# Autodesk Inventor assembly: Rwing
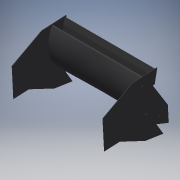
[picture p0: Inventor's stored thumbnail of the model, 180x180]
Saved by Autodesk Inventor 2018.2 (Build 222227000, 227)
## iProperties
Created: 2017-12-28
Part Number: Rwing
Material: 一般
Document SubType Name: Assembly
Designer: formula
Author: formula
## Documents named in this file (5)
- Z:\各班フォルダ\2018\ボディ\カウル\AeroCAD2018\CAD\Inventor\解析用CAD\R-wing\Rwing.iam
- Z:\各班フォルダ\2018\ボディ\カウル\AeroCAD2018\CAD\Inventor\解析用CAD\R-wing\parts\main_flap\parts\styro_50_main_center.ipt
- Z:\各班フォルダ\2018\ボディ\カウル\AeroCAD2018\CAD\Inventor\解析用CAD\R-wing\parts\sub_flap\parts\styro_50_sub.ipt
- Z:\各班フォルダ\2018\ボディ\カウル\AeroCAD2018\CAD\Inventor\解析用CAD\R-wing\parts\end_plate.ipt
- Z:\各班フォルダ\2018\ボディ\カウル\AeroCAD2018\CAD\Inventor\解析用CAD\R-wing\parts\foward_flap.ipt
## Components (5 placed, 4 different names)
1. styro_50_main_center:1 — メイト:1, メイト:2, メイト:3, メイト:4, メイト:5, メイト:6
2. styro_50_sub:1 — メイト:7, メイト:8, メイト:9
3. end_plate:1 — メイト:1, メイト:2, メイト:6, メイト:7, メイト:8, 角度:1
4. end_plate:2 — メイト:3, メイト:4, メイト:5, メイト:9, メイト:10, フラッシュ:1
5. foward_flap:1 — 角度:1, メイト:10, フラッシュ:1
## Relationships (12: Mate 10, Angle 1, Flush 1)
- メイト:1 [Mate]: styro_50_main_center:1 ↔ end_plate:1
- メイト:2 [Mate]: styro_50_main_center:1 ↔ end_plate:1
- メイト:3 [Mate]: styro_50_main_center:1 ↔ end_plate:2
- メイト:4 [Mate]: styro_50_main_center:1 ↔ end_plate:2
- メイト:5 [Mate]: styro_50_main_center:1 ↔ end_plate:2
- メイト:6 [Mate]: styro_50_main_center:1 ↔ end_plate:1
- メイト:7 [Mate]: styro_50_sub:1 ↔ end_plate:1
- メイト:8 [Mate]: styro_50_sub:1 ↔ end_plate:1
- メイト:9 [Mate]: styro_50_sub:1 ↔ end_plate:2
- 角度:1 [Angle] (0 deg): end_plate:1 ↔ foward_flap:1
- メイト:10 [Mate]: end_plate:2 ↔ foward_flap:1
- フラッシュ:1 [Flush] (10 mm): end_plate:2 ↔ foward_flap:1
